# Autodesk Inventor assembly: 001_light_all
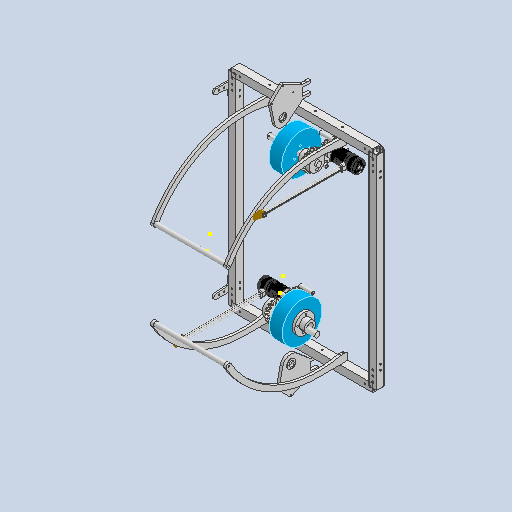
[picture p0: Inventor's stored thumbnail of the model, 512x512]
Saved by Autodesk Inventor 2025.2 (Build 292293000, 293)
## iProperties
Created: 2025-05-06
Part Number: 001_light_all
Document SubType Name: Assembly
Designer: yuki0520
Author: yuki0520
## Documents named in this file (7)
- C:\Users\haruy\Documents\ロボコン\NHK2025\cad\nagahisa\tanaka_dribll\2025_nhk\01\001_light_all.iam
- C:\Users\haruy\Documents\ロボコン\NHK2025\cad\nagahisa\tanaka_dribll\2025_nhk\01\01_light_wheel.iam
- C:\Users\haruy\Documents\ロボコン\NHK2025\cad\nagahisa\tanaka_dribll\2025_nhk\01\light_kaku_connect.ipt
- C:\Users\haruy\Documents\ロボコン\NHK2025\cad\nagahisa\tanaka_dribll\2025_nhk\tanaka\nageru\smallring\kakutome_nc.ipt
- C:\Users\haruy\Documents\ロボコン\NHK2025\cad\nagahisa\tanaka_dribll\2025_nhk\01\light_ball_space_nc.ipt
- C:\Users\haruy\Documents\ロボコン\NHK2025\cad\nagahisa\tanaka_dribll\2025_nhk\01\light_ball_space_side.ipt
- C:\Users\haruy\Documents\ロボコン\NHK2025\cad\nagahisa\tanaka_dribll\2025_nhk\01\light_ball_space_pole.ipt
## Components (16 placed, 6 different names)
1. 01_light_wheel:1 [sub-assembly] — 挿入:9, 挿入:10, 挿入:11, 挿入:12, 挿入:36, 挿入:37
2. 01_light_wheel:2 [sub-assembly] — 挿入:13, 挿入:14, 挿入:32, 挿入:33
3. light_kaku_connect:1 — 挿入:3, 挿入:4, 挿入:7, 挿入:8, 挿入:18, 挿入:20, 挿入:28, 挿入:29
4. light_kaku_connect:2 — 挿入:1, 挿入:2, 挿入:5, 挿入:6
5. kakutome_nc:1 — 挿入:7, 挿入:8, 挿入:9, 挿入:10
6. kakutome_nc:2 — 挿入:3, 挿入:4
7. kakutome_nc:3 — 挿入:5, 挿入:6, 挿入:13, 挿入:14
8. kakutome_nc:4 — 挿入:1, 挿入:2, 挿入:11, 挿入:12
9. light_ball_space_nc:2 — 挿入:18, 挿入:29
10. light_ball_space_nc:4 — 挿入:20, 挿入:28
11. light_ball_space_side:1 — 挿入:32, 挿入:34
12. light_ball_space_side:2 — 挿入:33, メイト:1
13. light_ball_space_pole:1 — 挿入:34, メイト:1
14. light_ball_space_side:3 — 挿入:37, メイト:2
15. light_ball_space_side:4 — 挿入:36, 挿入:38
16. light_ball_space_pole:2 — 挿入:38, メイト:2
## Relationships (26: Insert 24, Mate 2)
- 挿入:1 [Insert]: light_kaku_connect:2 ↔ kakutome_nc:4
- 挿入:2 [Insert]: light_kaku_connect:2 ↔ kakutome_nc:4
- 挿入:3 [Insert]: light_kaku_connect:1 ↔ kakutome_nc:2
- 挿入:4 [Insert]: light_kaku_connect:1 ↔ kakutome_nc:2
- 挿入:5 [Insert]: light_kaku_connect:2 ↔ kakutome_nc:3
- 挿入:6 [Insert]: light_kaku_connect:2 ↔ kakutome_nc:3
- 挿入:7 [Insert]: light_kaku_connect:1 ↔ kakutome_nc:1
- 挿入:8 [Insert]: light_kaku_connect:1 ↔ kakutome_nc:1
- 挿入:9 [Insert]: 01_light_wheel:1 ↔ kakutome_nc:1
- 挿入:10 [Insert]: 01_light_wheel:1 ↔ kakutome_nc:1
- 挿入:11 [Insert]: 01_light_wheel:1 ↔ kakutome_nc:4
- 挿入:12 [Insert]: 01_light_wheel:1 ↔ kakutome_nc:4
- 挿入:13 [Insert]: 01_light_wheel:2 ↔ kakutome_nc:3
- 挿入:14 [Insert]: 01_light_wheel:2 ↔ kakutome_nc:3
- 挿入:18 [Insert]: light_kaku_connect:1 ↔ light_ball_space_nc:2
- 挿入:20 [Insert]: light_kaku_connect:1 ↔ light_ball_space_nc:4
- 挿入:28 [Insert]: light_kaku_connect:1 ↔ light_ball_space_nc:4
- 挿入:29 [Insert]: light_kaku_connect:1 ↔ light_ball_space_nc:2
- 挿入:32 [Insert]: 01_light_wheel:2 ↔ light_ball_space_side:1
- 挿入:33 [Insert]: 01_light_wheel:2 ↔ light_ball_space_side:2
- 挿入:34 [Insert]: light_ball_space_side:1 ↔ light_ball_space_pole:1
- メイト:1 [Mate]: light_ball_space_side:2 ↔ light_ball_space_pole:1
- 挿入:36 [Insert]: 01_light_wheel:1 ↔ light_ball_space_side:4
- 挿入:37 [Insert]: 01_light_wheel:1 ↔ light_ball_space_side:3
- 挿入:38 [Insert]: light_ball_space_side:4 ↔ light_ball_space_pole:2
- メイト:2 [Mate]: light_ball_space_side:3 ↔ light_ball_space_pole:2
